# Autodesk Inventor assembly: External Frame
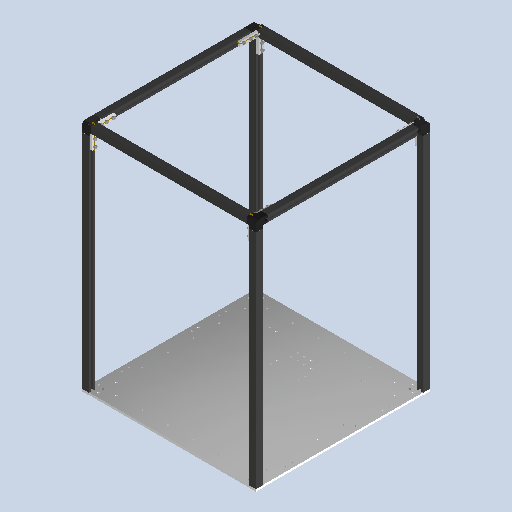
[picture p0: Inventor's stored thumbnail of the model, 512x512]
Saved by Autodesk Inventor 2024 (Build 280153000, 153)
## iProperties
Created: 2024-11-09
Part Number: External Frame
Document SubType Name: Assembly
Designer: Ishaan
Author: Ishaan
## Documents named in this file (13)
- E:\Projects\Axiom--IDEX-3D-Printer\CAD\02 - Frame\External Frame.iam
- E:\Projects\Axiom--IDEX-3D-Printer\CAD\02 - Frame\Printer Base Plate RevII.ipt
- E:\Projects\Axiom--IDEX-3D-Printer\CAD\00 - COTS Components\2020 Frame Exterior Corners\HFSTB5-2020-650.ipt
- E:\Projects\Axiom--IDEX-3D-Printer\CAD\08 - Side Panelling\Exterior Frame Corner Other.ipt
- E:\Projects\Axiom--IDEX-3D-Printer\CAD\08 - Side Panelling\Exterior Frame Corner.ipt
- E:\Projects\Axiom--IDEX-3D-Printer\CAD\00 - COTS Components\2020 Frame Exterior Y Runners\HFSFB5-2020-440.ipt
- E:\Projects\Axiom--IDEX-3D-Printer\CAD\08 - Side Panelling\Top Corner Extrusion Plate.ipt
- E:\Projects\Axiom--IDEX-3D-Printer\CAD\00 - COTS Components\2020 Frame Exterior X Runners\HFSTB5-2020-456.ipt
- E:\Projects\Axiom--IDEX-3D-Printer\CAD\00 - COTS Components\Hardware\SHCSM5x12.ipt
- E:\Projects\Axiom--IDEX-3D-Printer\CAD\00 - COTS Components\Hardware\SHCSM5x16.ipt
- E:\Projects\Axiom--IDEX-3D-Printer\CAD\00 - COTS Components\Hardware\M5 LOCKNUT.ipt
- E:\Projects\Axiom--IDEX-3D-Printer\CAD\00 - COTS Components\Hardware\M5 T SLOT NUT.ipt
- E:\Projects\Axiom--IDEX-3D-Printer\CAD\00 - COTS Components\Hardware\Low Profile M5x12.ipt
## Components (65 placed, 12 different names)
1. Printer Base Plate RevII:1 — Insert:1, Insert:2, Insert:3, Insert:4, Insert:57, Insert:58, Insert:59, Insert:60
2. HFSTB5-2020-650:1 — Insert:4, Flush:10, Flush:11, Mate:6
3. HFSTB5-2020-650:2 — Insert:3, Flush:2, Mate:1
4. HFSTB5-2020-650:3 — Insert:1, Flush:3, Flush:4, Mate:2
5. HFSTB5-2020-650:4 — Insert:2, Flush:8, Flush:9, Mate:5
6. Exterior Frame Corner Other:1 — Flush:8, Flush:9, Mate:5, Mate:8, Flush:14, Flush:15, Insert:5, Mate:9, Flush:16, Insert:18, Angle:2
7. Exterior Frame Corner:1 — Flush:3, Flush:4, Mate:2, Flush:5, Flush:6, Mate:3, Insert:8, Mate:12, Insert:52, Angle:17
8. Exterior Frame Corner Other:2 — Flush:2, Mate:1, Flush:7, Mate:4, Insert:7, Mate:11, Insert:42, Angle:12
9. Exterior Frame Corner:2 — Flush:10, Flush:11, Mate:6, Mate:7, Flush:12, Flush:13, Insert:6, Mate:10, Angle:1, Insert:32, Angle:7
10. HFSFB5-2020-440:1 — Flush:5, Flush:6, Flush:7, Mate:3, Mate:4
11. HFSFB5-2020-440:2 — Mate:7, Flush:12, Flush:13, Mate:8, Flush:14, Flush:15
12. Top Corner Extrusion Plate:1 — Insert:5, Mate:9, Insert:12, Insert:13, Insert:14, Insert:15, Insert:16, Insert:17, Insert:19, Insert:20, Insert:21, Insert:22, Angle:3, Angle:4, Angle:5, Angle:6, Insert:56
13. Top Corner Extrusion Plate:2 — Insert:6, Mate:10, Insert:9, Insert:23, Insert:24, Insert:25, Insert:26, Insert:27, Insert:28, Insert:29, Insert:30, Insert:31, Angle:8, Angle:9, Angle:10, Angle:11, Insert:53
14. Top Corner Extrusion Plate:3 — Insert:7, Mate:11, Insert:10, Insert:33, Insert:34, Insert:35, Insert:36, Insert:37, Insert:38, Insert:39, Insert:40, Insert:41, Angle:13, Angle:14, Angle:15, Angle:16, Insert:54
15. Top Corner Extrusion Plate:4 — Insert:8, Mate:12, Insert:11, Insert:43, Insert:44, Insert:45, Insert:46, Insert:47, Insert:48, Insert:49, Insert:50, Insert:51, Angle:18, Angle:19, Angle:20, Angle:21, Insert:55
16. HFSTB5-2020-456:1 — Insert:9, Angle:1, Insert:10
17. HFSTB5-2020-456:2 — Insert:11, Insert:12, Flush:16
18. Low Profile M5x12:1 — Insert:59
19. Low Profile M5x12:2 — Insert:60
20. Low Profile M5x12:3 — Insert:58
21. Low Profile M5x12:4 — Insert:57
22. SHCSM5x12:1 — Insert:13
23. SHCSM5x12:2 — Insert:14
24. SHCSM5x12:3 — Insert:15
25. SHCSM5x12:4 — Insert:16
26. SHCSM5x16:1 — Insert:17
27. M5 LOCKNUT:1 — Insert:18, Angle:2
28. M5 T SLOT NUT:1 — Insert:21, Angle:3
29. M5 T SLOT NUT:2 — Insert:19, Angle:6
30. M5 T SLOT NUT:3 — Insert:20, Angle:5
31. M5 T SLOT NUT:4 — Insert:22, Angle:4
32. SHCSM5x12:5 — Insert:27
33. SHCSM5x12:6 — Insert:26
34. SHCSM5x12:7 — Insert:23
35. SHCSM5x12:8 — Insert:24
36. SHCSM5x16:2 — Insert:25
37. M5 LOCKNUT:2 — Insert:32, Angle:7
38. M5 T SLOT NUT:5 — Insert:28, Angle:10
39. M5 T SLOT NUT:6 — Insert:30, Angle:8
40. M5 T SLOT NUT:7 — Insert:31, Angle:9
41. M5 T SLOT NUT:8 — Insert:29, Angle:11
42. SHCSM5x12:9 — Insert:33
43. SHCSM5x12:10 — Insert:34
44. SHCSM5x12:11 — Insert:36
45. SHCSM5x12:12 — Insert:37
46. SHCSM5x16:3 — Insert:35
47. M5 LOCKNUT:3 — Insert:42, Angle:12
48. M5 T SLOT NUT:9 — Insert:38, Angle:15
49. M5 T SLOT NUT:10 — Insert:41, Angle:14
50. M5 T SLOT NUT:11 — Insert:40, Angle:13
51. M5 T SLOT NUT:12 — Insert:39, Angle:16
52. SHCSM5x12:13 — Insert:47
53. SHCSM5x12:14 — Insert:46
54. SHCSM5x12:15 — Insert:43
55. SHCSM5x12:16 — Insert:44
56. SHCSM5x16:4 — Insert:45
57. M5 LOCKNUT:4 — Insert:52, Angle:17
58. M5 T SLOT NUT:13 — Insert:49, Angle:20
59. M5 T SLOT NUT:14 — Insert:50, Angle:18
60. M5 T SLOT NUT:15 — Insert:51, Angle:19
61. M5 T SLOT NUT:16 — Insert:48, Angle:21
62. SHCSM5x16:5 — Insert:53
63. SHCSM5x16:6 — Insert:54
64. SHCSM5x16:7 — Insert:56
65. SHCSM5x16:8 — Insert:55
## Relationships (108: Insert 60, Angle 21, Flush 15, Mate 12)
- Insert:1: Printer Base Plate RevII:1 ↔ HFSTB5-2020-650:3
- Insert:2: Printer Base Plate RevII:1 ↔ HFSTB5-2020-650:4
- Insert:3: Printer Base Plate RevII:1 ↔ HFSTB5-2020-650:2
- Insert:4: Printer Base Plate RevII:1 ↔ HFSTB5-2020-650:1
- Flush:2: HFSTB5-2020-650:2 ↔ Exterior Frame Corner Other:2
- Mate:1 (0.2 mm): HFSTB5-2020-650:2 ↔ Exterior Frame Corner Other:2
- Flush:3: HFSTB5-2020-650:3 ↔ Exterior Frame Corner:1
- Flush:4: HFSTB5-2020-650:3 ↔ Exterior Frame Corner:1
- Mate:2 (0.2 mm): HFSTB5-2020-650:3 ↔ Exterior Frame Corner:1
- Flush:5: Exterior Frame Corner:1 ↔ HFSFB5-2020-440:1
- Flush:6: Exterior Frame Corner:1 ↔ HFSFB5-2020-440:1
- Flush:7: Exterior Frame Corner Other:2 ↔ HFSFB5-2020-440:1
- Mate:3 (0.2 mm): Exterior Frame Corner:1 ↔ HFSFB5-2020-440:1
- Mate:4 (0.2 mm): Exterior Frame Corner Other:2 ↔ HFSFB5-2020-440:1
- Flush:8: HFSTB5-2020-650:4 ↔ Exterior Frame Corner Other:1
- Flush:9: HFSTB5-2020-650:4 ↔ Exterior Frame Corner Other:1
- Mate:5 (0.2 mm): HFSTB5-2020-650:4 ↔ Exterior Frame Corner Other:1
- Flush:10: HFSTB5-2020-650:1 ↔ Exterior Frame Corner:2
- Flush:11: HFSTB5-2020-650:1 ↔ Exterior Frame Corner:2
- Mate:6 (0.2 mm): HFSTB5-2020-650:1 ↔ Exterior Frame Corner:2
- Mate:7 (0.2 mm): Exterior Frame Corner:2 ↔ HFSFB5-2020-440:2
- Flush:12: Exterior Frame Corner:2 ↔ HFSFB5-2020-440:2
- Flush:13: Exterior Frame Corner:2 ↔ HFSFB5-2020-440:2
- Mate:8 (0.2 mm): Exterior Frame Corner Other:1 ↔ HFSFB5-2020-440:2
- Flush:14: Exterior Frame Corner Other:1 ↔ HFSFB5-2020-440:2
- Flush:15: Exterior Frame Corner Other:1 ↔ HFSFB5-2020-440:2
- Insert:5: Exterior Frame Corner Other:1 ↔ Top Corner Extrusion Plate:1
- Mate:9: Exterior Frame Corner Other:1 ↔ Top Corner Extrusion Plate:1
- Insert:6: Exterior Frame Corner:2 ↔ Top Corner Extrusion Plate:2
- Mate:10: Exterior Frame Corner:2 ↔ Top Corner Extrusion Plate:2
- Insert:7: Exterior Frame Corner Other:2 ↔ Top Corner Extrusion Plate:3
- Mate:11: Exterior Frame Corner Other:2 ↔ Top Corner Extrusion Plate:3
- Insert:8: Exterior Frame Corner:1 ↔ Top Corner Extrusion Plate:4
- Mate:12: Exterior Frame Corner:1 ↔ Top Corner Extrusion Plate:4
- Insert:9: Top Corner Extrusion Plate:2 ↔ HFSTB5-2020-456:1
- Angle:1 (0 deg): Exterior Frame Corner:2 ↔ HFSTB5-2020-456:1
- Insert:10: Top Corner Extrusion Plate:3 ↔ HFSTB5-2020-456:1
- Insert:11: Top Corner Extrusion Plate:4 ↔ HFSTB5-2020-456:2
- Insert:12: Top Corner Extrusion Plate:1 ↔ HFSTB5-2020-456:2
- Flush:16: Exterior Frame Corner Other:1 ↔ HFSTB5-2020-456:2
- Insert:13: Top Corner Extrusion Plate:1 ↔ SHCSM5x12:1
- Insert:14: Top Corner Extrusion Plate:1 ↔ SHCSM5x12:2
- Insert:15: Top Corner Extrusion Plate:1 ↔ SHCSM5x12:3
- Insert:16: Top Corner Extrusion Plate:1 ↔ SHCSM5x12:4
- Insert:17: Top Corner Extrusion Plate:1 ↔ SHCSM5x16:1
- Insert:18: Exterior Frame Corner Other:1 ↔ M5 LOCKNUT:1
- Angle:2 (0 deg): Exterior Frame Corner Other:1 ↔ M5 LOCKNUT:1
- Insert:19 (2 mm): Top Corner Extrusion Plate:1 ↔ M5 T SLOT NUT:2
- Insert:20 (2 mm): Top Corner Extrusion Plate:1 ↔ M5 T SLOT NUT:3
- Insert:21 (2 mm): Top Corner Extrusion Plate:1 ↔ M5 T SLOT NUT:1
- Insert:22 (2 mm): Top Corner Extrusion Plate:1 ↔ M5 T SLOT NUT:4
- Angle:3 (0 deg): Top Corner Extrusion Plate:1 ↔ M5 T SLOT NUT:1
- Angle:4 (0 deg): Top Corner Extrusion Plate:1 ↔ M5 T SLOT NUT:4
- Angle:5 (0 deg): Top Corner Extrusion Plate:1 ↔ M5 T SLOT NUT:3
- Angle:6 (0 deg): Top Corner Extrusion Plate:1 ↔ M5 T SLOT NUT:2
- Insert:23: Top Corner Extrusion Plate:2 ↔ SHCSM5x12:7
- Insert:24: Top Corner Extrusion Plate:2 ↔ SHCSM5x12:8
- Insert:25: Top Corner Extrusion Plate:2 ↔ SHCSM5x16:2
- Insert:26: Top Corner Extrusion Plate:2 ↔ SHCSM5x12:6
- Insert:27: Top Corner Extrusion Plate:2 ↔ SHCSM5x12:5
- Insert:28 (2 mm): Top Corner Extrusion Plate:2 ↔ M5 T SLOT NUT:5
- Insert:29 (2 mm): Top Corner Extrusion Plate:2 ↔ M5 T SLOT NUT:8
- Insert:30 (2 mm): Top Corner Extrusion Plate:2 ↔ M5 T SLOT NUT:6
- Insert:31 (2 mm): Top Corner Extrusion Plate:2 ↔ M5 T SLOT NUT:7
- Insert:32: Exterior Frame Corner:2 ↔ M5 LOCKNUT:2
- Angle:7 (0 deg): Exterior Frame Corner:2 ↔ M5 LOCKNUT:2
- Angle:8 (0 deg): Top Corner Extrusion Plate:2 ↔ M5 T SLOT NUT:6
- Angle:9 (0 deg): Top Corner Extrusion Plate:2 ↔ M5 T SLOT NUT:7
- Angle:10 (0 deg): Top Corner Extrusion Plate:2 ↔ M5 T SLOT NUT:5
- Angle:11 (0 deg): Top Corner Extrusion Plate:2 ↔ M5 T SLOT NUT:8
- Insert:33: Top Corner Extrusion Plate:3 ↔ SHCSM5x12:9
- Insert:34: Top Corner Extrusion Plate:3 ↔ SHCSM5x12:10
- Insert:35: Top Corner Extrusion Plate:3 ↔ SHCSM5x16:3
- Insert:36: Top Corner Extrusion Plate:3 ↔ SHCSM5x12:11
- Insert:37: Top Corner Extrusion Plate:3 ↔ SHCSM5x12:12
- Insert:38 (2 mm): Top Corner Extrusion Plate:3 ↔ M5 T SLOT NUT:9
- Insert:39 (2 mm): Top Corner Extrusion Plate:3 ↔ M5 T SLOT NUT:12
- Insert:40 (2 mm): Top Corner Extrusion Plate:3 ↔ M5 T SLOT NUT:11
- Insert:41 (2 mm): Top Corner Extrusion Plate:3 ↔ M5 T SLOT NUT:10
- Insert:42: Exterior Frame Corner Other:2 ↔ M5 LOCKNUT:3
- Angle:12 (0 deg): Exterior Frame Corner Other:2 ↔ M5 LOCKNUT:3
- Angle:13 (0 deg): Top Corner Extrusion Plate:3 ↔ M5 T SLOT NUT:11
- Angle:14 (0 deg): Top Corner Extrusion Plate:3 ↔ M5 T SLOT NUT:10
- Angle:15 (0 deg): Top Corner Extrusion Plate:3 ↔ M5 T SLOT NUT:9
- Angle:16 (0 deg): Top Corner Extrusion Plate:3 ↔ M5 T SLOT NUT:12
- Insert:43: Top Corner Extrusion Plate:4 ↔ SHCSM5x12:15
- Insert:44: Top Corner Extrusion Plate:4 ↔ SHCSM5x12:16
- Insert:45: Top Corner Extrusion Plate:4 ↔ SHCSM5x16:4
- Insert:46: Top Corner Extrusion Plate:4 ↔ SHCSM5x12:14
- Insert:47: Top Corner Extrusion Plate:4 ↔ SHCSM5x12:13
- Insert:48 (2 mm): Top Corner Extrusion Plate:4 ↔ M5 T SLOT NUT:16
- Insert:49 (2 mm): Top Corner Extrusion Plate:4 ↔ M5 T SLOT NUT:13
- Insert:50 (2 mm): Top Corner Extrusion Plate:4 ↔ M5 T SLOT NUT:14
- Insert:51 (2 mm): Top Corner Extrusion Plate:4 ↔ M5 T SLOT NUT:15
- Insert:52: Exterior Frame Corner:1 ↔ M5 LOCKNUT:4
- Angle:17 (0 deg): Exterior Frame Corner:1 ↔ M5 LOCKNUT:4
- Angle:18 (0 deg): Top Corner Extrusion Plate:4 ↔ M5 T SLOT NUT:14
- Angle:19 (0 deg): Top Corner Extrusion Plate:4 ↔ M5 T SLOT NUT:15
- Angle:20 (0 deg): Top Corner Extrusion Plate:4 ↔ M5 T SLOT NUT:13
- Angle:21 (0 deg): Top Corner Extrusion Plate:4 ↔ M5 T SLOT NUT:16
- Insert:53: Top Corner Extrusion Plate:2 ↔ SHCSM5x16:5
- Insert:54: Top Corner Extrusion Plate:3 ↔ SHCSM5x16:6
- Insert:55: Top Corner Extrusion Plate:4 ↔ SHCSM5x16:8
- Insert:56: Top Corner Extrusion Plate:1 ↔ SHCSM5x16:7
- Insert:57: Printer Base Plate RevII:1 ↔ Low Profile M5x12:4
- Insert:58: Printer Base Plate RevII:1 ↔ Low Profile M5x12:3
- Insert:59: Printer Base Plate RevII:1 ↔ Low Profile M5x12:1
- Insert:60: Printer Base Plate RevII:1 ↔ Low Profile M5x12:2
